# Autodesk Inventor assembly: Extruder
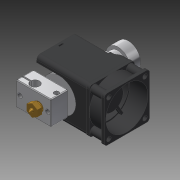
[picture p0: Inventor's stored thumbnail of the model, 180x180]
Saved by Autodesk Inventor 2014 SP1 (Build 180222100, 222)
## iProperties
Created: 2017-12-02
Part Number: Extruder
Document SubType Name: Assembly
Designer: Stepan
Author: Stepan
## Documents named in this file (4)
- D:\3DPrinter\Extruder.iam
- D:\3DPrinter\Hot-end\HOT-END.iam
- D:\3DPrinter\Plastic_Details\COOLER-HOLDER.ipt
- D:\3DPrinter\Cooler\Cooler.ipt
## Components (3 placed, 3 different names)
1. HOT-END:1 [sub-assembly] — Совмещение:1, Заподлицо:1, Заподлицо:4
2. COOLER-HOLDER:1 — Совмещение:1, Заподлицо:1, Совмещение:2, Заподлицо:2, Заподлицо:3, Заподлицо:4
3. Cooler:1 — Совмещение:2, Заподлицо:2, Заподлицо:3
## Relationships (6: Flush 4, Mate 2)
- Совмещение:1 [Mate]: HOT-END:1 ↔ COOLER-HOLDER:1
- Заподлицо:1 [Flush]: HOT-END:1 ↔ COOLER-HOLDER:1
- Совмещение:2 [Mate]: COOLER-HOLDER:1 ↔ Cooler:1
- Заподлицо:2 [Flush]: COOLER-HOLDER:1 ↔ Cooler:1
- Заподлицо:3 [Flush]: COOLER-HOLDER:1 ↔ Cooler:1
- Заподлицо:4 [Flush]: HOT-END:1 ↔ COOLER-HOLDER:1
